# Autodesk Inventor assembly: Output_bearing_assembly
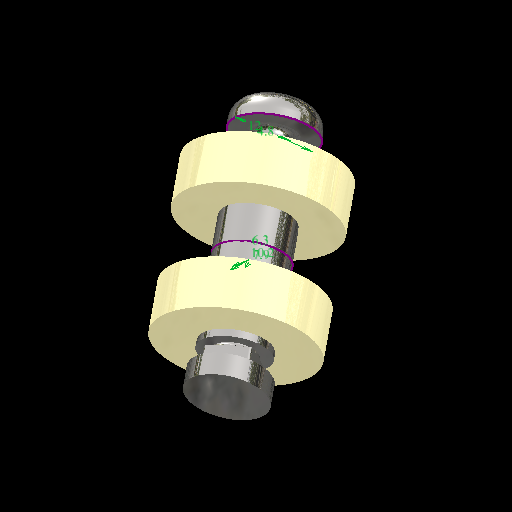
[picture p0: Inventor's stored thumbnail of the model, 512x512]
Saved by Autodesk Inventor 2022.2 (Build 262287010, 287A)
## iProperties
Created: 2022-05-10
Part Number: Output_bearing_assembly
Document SubType Name: Assembly
Designer: Árni Þór Þorgeirsson
Author: Árni Þór Þorgeirsson
## Documents named in this file (6)
- G:\My Drive\Masters Thesis - exo\CAD_Files\External Hardware\Output_bearing_assembly.iam
- G:\My Drive\Masters Thesis - exo\CAD_Files\External Hardware\608 bearing.ipt
- G:\My Drive\Masters Thesis - exo\CAD_Files\External Hardware\brushing.ipt
- G:\My Drive\Masters Thesis - exo\CAD_Files\External Hardware\skaterScrew.ipt
- G:\My Drive\Masters Thesis - exo\CAD_Files\External Hardware\spacer.ipt
- G:\My Drive\Masters Thesis - exo\CAD_Files\External Hardware\SkaterInsertScrew.ipt
## Components (7 placed, 5 different names)
1. 608 bearing:2 — Insert:1, Insert:4
2. brushing:1 — Insert:4, Insert:6
3. skaterScrew:1 — Insert:5
4. spacer:1 — Insert:1, Insert:2
5. 608 bearing:3 — Insert:2, Insert:3
6. brushing:2 — Insert:3, Insert:5
7. SkaterInsertScrew:1 — Insert:6
## Relationships (6: Insert 6)
- Insert:1: 608 bearing:2 ↔ spacer:1
- Insert:2: spacer:1 ↔ 608 bearing:3
- Insert:3: 608 bearing:3 ↔ brushing:2
- Insert:4: 608 bearing:2 ↔ brushing:1
- Insert:5: skaterScrew:1 ↔ brushing:2
- Insert:6 (-3 mm): brushing:1 ↔ SkaterInsertScrew:1
